# Autodesk Inventor assembly: assembledLinkage
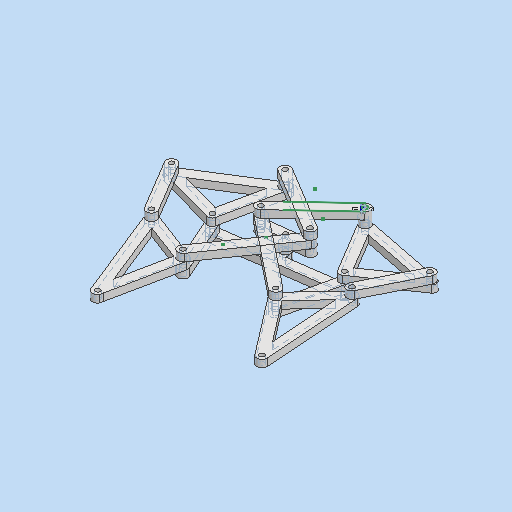
[picture p0: Inventor's stored thumbnail of the model, 512x512]
Saved by Autodesk Inventor 2026 (Build 300175000, 175)
## iProperties
Created: 2025-05-24
Part Number: assembledLinkage
Document SubType Name: Assembly
Designer: omiye
Author: omiye
## Documents named in this file (10)
- M:\strandbeest\assembledLinkage.iam
- M:\strandbeest\f.ipt
- M:\strandbeest\k.ipt
- M:\strandbeest\c.ipt
- M:\strandbeest\bde.ipt
- M:\strandbeest\ghi.ipt
- M:\strandbeest\m.ipt
- M:\strandbeest\j.ipt
- M:\strandbeest\connector.ipt
- M:\strandbeest\ghiMirror.ipt
## Components (14 placed, 9 different names)
1. f:1 — Mate:13, Mate:14, Mate:25, Mate:31
2. k:1 — Mate:2, Mate:5, Mate:16, Mate:23, Mate:27, Mate:30
3. c:1 — Mate:15, Mate:16, Mate:24, Mate:28, Mate:29
4. bde:1 — Mate:7, Mate:13, Mate:15, Flush:1, Mate:25, Mate:31
5. ghi:1 — Mate:5, Mate:14, Mate:23, Mate:24, Flush:1
6. m:1 — Mate:2, Mate:3, Mate:21, Mate:27, Mate:32, Mate:33
7. j:1 — Mate:3, Mate:7, Mate:30
8. connector:1 — Mate:21, Mate:28, Mate:29, Mate:40, Mate:43, Mate:52
9. bde:2 — Mate:39, Mate:40, Mate:41, Mate:54, Mate:56
10. c:2 — Mate:43, Mate:52, Mate:53
11. f:2 — Mate:54, Mate:55, Mate:56
12. j:2 — Mate:36, Mate:37, Mate:39, Mate:41
13. k:2 — Mate:32, Mate:33, Mate:36, Mate:37, Mate:47, Mate:51, Mate:53
14. ghiMirror:1 — Mate:47, Mate:51, Mate:55
## Relationships (33: Mate 32, Flush 1)
- Mate:2: k:1 ↔ m:1
- Mate:3: m:1 ↔ j:1
- Mate:5: k:1 ↔ ghi:1
- Mate:7: bde:1 ↔ j:1
- Mate:13: f:1 ↔ bde:1
- Mate:14: f:1 ↔ ghi:1
- Mate:15: c:1 ↔ bde:1
- Mate:16: k:1 ↔ c:1
- Mate:21: m:1 ↔ connector:1
- Mate:23: k:1 ↔ ghi:1
- Mate:24: c:1 ↔ ghi:1
- Flush:1: bde:1 ↔ ghi:1
- Mate:25: f:1 ↔ bde:1
- Mate:27: k:1 ↔ m:1
- Mate:28: c:1 ↔ connector:1
- Mate:29: c:1 ↔ connector:1
- Mate:30: k:1 ↔ j:1
- Mate:31: f:1 ↔ bde:1
- Mate:32: m:1 ↔ k:2
- Mate:33: m:1 ↔ k:2
- Mate:36: j:2 ↔ k:2
- Mate:37: j:2 ↔ k:2
- Mate:39: bde:2 ↔ j:2
- Mate:40: connector:1 ↔ bde:2
- Mate:41: bde:2 ↔ j:2
- Mate:43: connector:1 ↔ c:2
- Mate:47: k:2 ↔ ghiMirror:1
- Mate:51: k:2 ↔ ghiMirror:1
- Mate:52: connector:1 ↔ c:2
- Mate:53: c:2 ↔ k:2
- Mate:54: bde:2 ↔ f:2
- Mate:55: f:2 ↔ ghiMirror:1
- Mate:56: bde:2 ↔ f:2
